# Autodesk Inventor assembly: ringOuter_Split_Flat
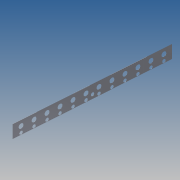
[picture p0: Inventor's stored thumbnail of the model, 180x180]
Saved by Autodesk Inventor 2014 SP1 (Build 180222100, 222)
## iProperties
Created: 2015-01-30
Part Number: ringOuter_Split_Flat
Document SubType Name: Assembly
Designer: Dave
Author: Dave
## Documents named in this file (3)
- C:\Users\Dave\Desktop\hera-cad\hub\ringOuter_Split_Flat.iam
- C:\Users\Dave\Desktop\hera-cad\hub\ringOuter_Split_Flat.ipt
- C:\Users\Dave\Desktop\hera-cad\hub\ringOuter_Split_Flat_MIR.ipt
## Components (2 placed, 2 different names)
1. ringOuter_Split_Flat:1 — Insert:1
2. ringOuter_Split_Flat_MIR:1 — Insert:1
## Relationships (1: Insert 1)
- Insert:1: ringOuter_Split_Flat:1 ↔ ringOuter_Split_Flat_MIR:1
